# Autodesk Inventor assembly: fab model mk-1
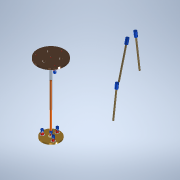
[picture p0: Inventor's stored thumbnail of the model, 180x180]
Saved by Autodesk Inventor 2020 (Build 240168000, 168)
## iProperties
Created: 2020-12-19
Part Number: fab model mk-1
Document SubType Name: Assembly
Designer: Vikki
Author: Vikki
## Documents named in this file (13)
- D:\borewell rescuebot\pll manipulator files\sps manipulator\fab model mk-2.iam
- D:\borewell rescuebot\pll manipulator files\sps manipulator\base.ipt
- D:\borewell rescuebot\pll manipulator files\sps manipulator\craftsman-3-pc-universal-joint-set-1.snapshot.1\Craftsman Socket U-Joint.iam
- D:\borewell rescuebot\pll manipulator files\sps manipulator\platform.ipt
- D:\borewell rescuebot\pll manipulator files\sps manipulator\leadscrew.ipt
- D:\borewell rescuebot\pll manipulator files\sps manipulator\coupler.ipt
- D:\borewell rescuebot\pll manipulator files\sps manipulator\telescopic boom1.ipt
- D:\borewell rescuebot\pll manipulator files\sps manipulator\boom 3.ipt
- D:\borewell rescuebot\pll manipulator files\sps manipulator\ball-pin.ipt
- D:\borewell rescuebot\2020 bot\borewell max sixe.ipt
- D:\borewell rescuebot\2020 bot\min size bore well.ipt
- D:\borewell rescuebot\pll manipulator files\sps manipulator\fab model mk-1\Design Accelerator\Bearing1.iam
- D:\borewell rescuebot\pll manipulator files\sps manipulator\connector plunger.ipt
## Components (26 placed, 12 different names)
1. base:1 — Mate:1, Mate:2, Mate:3, Mate:4, Mate:5, Mate:6, Angle:1, Mate:18, Mate:19, Mate:61, Flush:6, M1 C, M2 C
2. Craftsman Socket U-Joint:1 [sub-assembly] — Mate:1, Mate:2, Angle:2, Mate:25, Mate:90
3. Craftsman Socket U-Joint:2 [sub-assembly] — Mate:5, Mate:6, Angle:3, Mate:92
4. Craftsman Socket U-Joint:3 [sub-assembly] — Mate:3, Mate:4, Angle:1, Angle:2, Angle:3, Mate:23, Mate:91
5. platform:1 — Mate:7, Mate:8, Mate:9, Mate:10, Mate:11, Mate:12, Mate:16, Mate:17, Mate:63, Flush:8, Mate:64, Mate:65, Flush:9, Flush:10, M1 C, M2 C, Angle:6
6. Craftsman Socket U-Joint:4 [sub-assembly] — Mate:7, Mate:8, Mate:85, Mate:90
7. Craftsman Socket U-Joint:5 [sub-assembly] — Mate:9, Mate:12, Mate:25, Mate:86, Mate:88, Mate:91
8. Craftsman Socket U-Joint:6 [sub-assembly] — Mate:10, Mate:11, Mate:23, Mate:92
9. Craftsman Socket U-Joint:7 [sub-assembly] — Mate:16, Mate:17, Mate:26, Flush:1, Mate:52, Mate:60, Angle:6
10. Craftsman Socket U-Joint:8 [sub-assembly] — Mate:18, Mate:19, Angle:5, Mate:26, Flush:1, Mate:48, Mate:59
11. leadscrew:1 — Mate:37, Mate:38
12. coupler:1 — Mate:37, Mate:38
13. leadscrew:2
14. coupler:2
15. leadscrew:3
16. coupler:3
17. telescopic boom1:1 — Mate:48, Mate:51, Mate:59
18. boom 3:1 — Mate:51, Mate:52
19. ball-pin:1 — Mate:60
20. borewell max sixe:1 — Mate:61, Mate:62, Flush:5
21. min size bore well:1 — Mate:62, Flush:5, Flush:6
22. Bearing:1 [sub-assembly] — Mate:63, Flush:8
23. Bearing:2 [sub-assembly] — Mate:64, Flush:10
24. Bearing:3 [sub-assembly] — Mate:65, Flush:9
25. connector plunger:2 — Mate:86, Mate:88
26. connector plunger:3 — Mate:85
## Relationships (56: Mate 42, Flush 9, Angle 5)
- Mate:1: base:1 ↔ Craftsman Socket U-Joint:1
- Mate:2: base:1 ↔ Craftsman Socket U-Joint:1
- Mate:3: base:1 ↔ Craftsman Socket U-Joint:3
- Mate:4: base:1 ↔ Craftsman Socket U-Joint:3
- Mate:5: base:1 ↔ Craftsman Socket U-Joint:2
- Mate:6: base:1 ↔ Craftsman Socket U-Joint:2
- Mate:7: platform:1 ↔ Craftsman Socket U-Joint:4
- Mate:8: platform:1 ↔ Craftsman Socket U-Joint:4
- Mate:9: platform:1 ↔ Craftsman Socket U-Joint:5
- Mate:10: platform:1 ↔ Craftsman Socket U-Joint:6
- Mate:11: platform:1 ↔ Craftsman Socket U-Joint:6
- Mate:12: platform:1 ↔ Craftsman Socket U-Joint:5
- Angle:1 (30 deg): base:1 ↔ Craftsman Socket U-Joint:3
- Angle:2 (60 deg): Craftsman Socket U-Joint:1 ↔ Craftsman Socket U-Joint:3
- Angle:3 (120 deg): Craftsman Socket U-Joint:2 ↔ Craftsman Socket U-Joint:3
- Mate:16: platform:1 ↔ Craftsman Socket U-Joint:7
- Mate:17: platform:1 ↔ Craftsman Socket U-Joint:7
- Mate:18: base:1 ↔ Craftsman Socket U-Joint:8
- Mate:19: base:1 ↔ Craftsman Socket U-Joint:8
- Angle:5 (0 deg): Craftsman Socket U-Joint:8
- Mate:23: Craftsman Socket U-Joint:3 ↔ Craftsman Socket U-Joint:6
- Mate:25: Craftsman Socket U-Joint:1 ↔ Craftsman Socket U-Joint:5
- Mate:26: Craftsman Socket U-Joint:7 ↔ Craftsman Socket U-Joint:8
- Flush:1: Craftsman Socket U-Joint:7 ↔ Craftsman Socket U-Joint:8
- Mate:37: leadscrew:1 ↔ coupler:1
- Mate:38 (-10 mm): leadscrew:1 ↔ coupler:1
- [Mate]: leadscrew:2 ↔ coupler:2
- [Mate] (-10 mm): leadscrew:2 ↔ coupler:2
- [Mate]: leadscrew:3 ↔ coupler:3
- [Mate] (-10 mm): leadscrew:3 ↔ coupler:3
- Mate:48: Craftsman Socket U-Joint:8 ↔ telescopic boom1:1
- Mate:51: telescopic boom1:1 ↔ boom 3:1
- Mate:52: Craftsman Socket U-Joint:7 ↔ boom 3:1
- Mate:59 (-5 mm): Craftsman Socket U-Joint:8 ↔ telescopic boom1:1
- Mate:60: Craftsman Socket U-Joint:7 ↔ ball-pin:1
- [Flush]: borewell max sixe:1 ↔ min size bore well:1
- [Flush]: borewell max sixe:1 ↔ min size bore well:1
- Mate:61: base:1 ↔ borewell max sixe:1
- Mate:62: borewell max sixe:1 ↔ min size bore well:1
- Flush:5: borewell max sixe:1 ↔ min size bore well:1
- Flush:6 (-400 mm): base:1 ↔ min size bore well:1
- Mate:63: platform:1 ↔ Bearing:1
- Flush:8: platform:1 ↔ Bearing:1
- Mate:64: platform:1 ↔ Bearing:2
- Mate:65: platform:1 ↔ Bearing:3
- Flush:9: platform:1 ↔ Bearing:3
- Flush:10: platform:1 ↔ Bearing:2
- Mate:85 (0.5 mm): Craftsman Socket U-Joint:4 ↔ connector plunger:3
- Mate:86: Craftsman Socket U-Joint:5 ↔ connector plunger:2
- Mate:88 (0.5 mm): Craftsman Socket U-Joint:5 ↔ connector plunger:2
- M1 C [Flush] (400 mm): base:1 ↔ platform:1
- M2 C [Mate]: base:1 ↔ platform:1
- Mate:90: Craftsman Socket U-Joint:1 ↔ Craftsman Socket U-Joint:4
- Mate:91: Craftsman Socket U-Joint:3 ↔ Craftsman Socket U-Joint:5
- Mate:92: Craftsman Socket U-Joint:2 ↔ Craftsman Socket U-Joint:6
- Angle:6 (30 deg): platform:1 ↔ Craftsman Socket U-Joint:7
## Named parameters: d70_d68 = 0 mm, d71_d69 = -10 mm, d72_d68 = 0 mm, d73_d69 = -10 mm
